# Autodesk Inventor assembly: Gripper
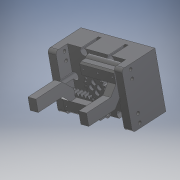
[picture p0: Inventor's stored thumbnail of the model, 180x180]
Saved by Autodesk Inventor 2017 (Build 210142000, 142)
## iProperties
Created: 2018-10-23
Part Number: Gripper
Document SubType Name: Assembly
Designer: Dell
Author: Dell
## Documents named in this file (6)
- C:\Users\Dell\Documents\GitHub\tr2\Gripper\Gripper.iam
- C:\Users\Dell\Documents\GitHub\tr2\Gripper\AX-12A.ipt
- C:\Users\Dell\Documents\GitHub\tr2\Gripper\Gripper\Design Accelerator\Spur Gears1.iam
- C:\Users\Dell\Documents\GitHub\tr2\Gripper\GA04.ipt
- C:\Users\Dell\Documents\GitHub\tr2\Gripper\GA01b.ipt
- C:\Users\Dell\Documents\GitHub\tr2\Gripper\GA05.ipt
## Components (7 placed, 5 different names)
1. GA01b:1 — Mate:24, Mate:25, Mate:26, Mate:28, Mate:29, Mate:30, Mate:31
2. AX-12A:2 — Mate:24, Mate:25, Mate:26, Mate:40
3. GA04:3 — Mate:28, Rotation/Translation:3, Mate:33, Mate:34, Mate:38
4. GA04:4 — Mate:29, Mate:30, Rotation/Translation:4, Mate:35, Mate:37, Mate:39
5. Spur Gears:2 [sub-assembly] — Mate:31, Rotation/Translation:3, Rotation/Translation:4, Mate:40
6. GA05:1 — Mate:33, Mate:34, Mate:38
7. GA05:2 — Mate:35, Mate:37, Mate:39
## Relationships (16: Mate 14, RelateRotateTranslate 2)
- Mate:24: GA01b:1 ↔ AX-12A:2
- Mate:25: GA01b:1 ↔ AX-12A:2
- Mate:26: GA01b:1 ↔ AX-12A:2
- Mate:28: GA01b:1 ↔ GA04:3
- Mate:29: GA01b:1 ↔ GA04:4
- Mate:30: GA01b:1 ↔ GA04:4
- Mate:31: GA01b:1 ↔ Spur Gears:2
- Rotation/Translation:3 [RelateRotateTranslate] (131 mm): GA04:3 ↔ Spur Gears:2
- Rotation/Translation:4 [RelateRotateTranslate] (131 mm): GA04:4 ↔ Spur Gears:2
- Mate:33: GA04:3 ↔ GA05:1
- Mate:34: GA04:3 ↔ GA05:1
- Mate:35: GA04:4 ↔ GA05:2
- Mate:37: GA04:4 ↔ GA05:2
- Mate:38: GA04:3 ↔ GA05:1
- Mate:39: GA04:4 ↔ GA05:2
- Mate:40: AX-12A:2 ↔ Spur Gears:2
